# Autodesk Inventor assembly: FINGER_asm
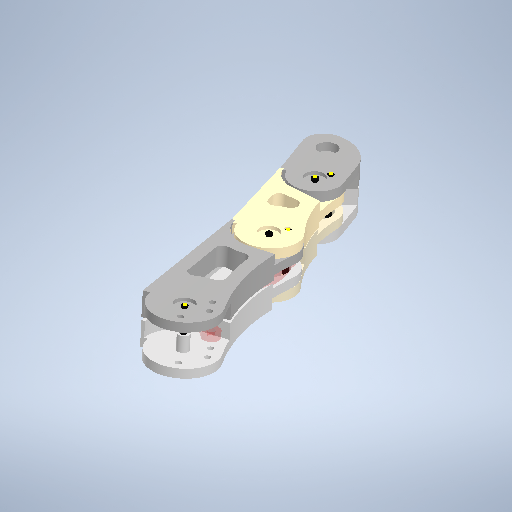
[picture p0: Inventor's stored thumbnail of the model, 512x512]
Saved by Autodesk Inventor 2025.2 (Build 292293000, 293)
## iProperties
Created: 2024-11-09
Part Number: FINGER_asm
Document SubType Name: Assembly
Designer: esandor
Author: esandor
## Documents named in this file (11)
- C:\Users\esandor\Documents\Inventor\Workspace\LEGO_GITHUB_INDACT_CAD\FINGER\FINGER_asm.iam
- C:\Users\esandor\Documents\Inventor\Workspace\LEGO_GITHUB_INDACT_CAD\FINGER\FIN_PD_B.ipt
- C:\Users\esandor\Documents\Inventor\Workspace\LEGO_GITHUB_INDACT_CAD\FINGER\FIN_PM_B.ipt
- C:\Users\esandor\Documents\Inventor\Workspace\LEGO_GITHUB_INDACT_CAD\FINGER\FIN_PP_B.ipt
- C:\Users\esandor\Documents\Inventor\Workspace\LEGO_GITHUB_INDACT_CAD\FINGER\FIN_PD_T.ipt
- C:\Users\esandor\Documents\Inventor\Workspace\LEGO_GITHUB_INDACT_CAD\FINGER\FIN_PM_T.ipt
- C:\Users\esandor\Documents\Inventor\Workspace\LEGO_GITHUB_INDACT_CAD\FINGER\FIN_DP_L.ipt
- C:\Users\esandor\Documents\Inventor\Workspace\LEGO_GITHUB_INDACT_CAD\FINGER\FIN_PP_T.ipt
- C:\Users\esandor\Documents\Inventor\Workspace\LEGO_GITHUB_INDACT_CAD\FINGER\FIN_DP_S.ipt
- C:\Users\esandor\Documents\Inventor\Workspace\LEGO_GITHUB_INDACT_CAD\FINGER\FIN_MD.ipt
- C:\Users\esandor\Documents\Inventor\Workspace\LEGO_GITHUB_INDACT_CAD\FINGER\FIN_MP.ipt
## Components (15 placed, 10 different names)
1. FIN_PD_B:1 — Mate:1, Rotational:1, Mate:3, Insert:1, Insert:2, Insert:5, Insert:9
2. FIN_PM_B:1 — Mate:1, Rotational:1, Insert:4, Rotational:2, Insert:10
3. FIN_PD_T:1 — Mate:3, Insert:1, Insert:2, Mate:4, Insert:3, Tangent:3
4. FIN_PM_T:1 — Mate:4, Insert:3, Tangent:1, Insert:6
5. FIN_DP_L:1 — Insert:4, Tangent:1
6. FIN_DP_L:2 — Insert:5, Insert:8
7. FIN_PP_B:1 — Rotational:2, Insert:7, Insert:11, Insert:12
8. FIN_PP_T:1 — Insert:6, Tangent:2, Mate:6, Tangent:6
9. FIN_DP_L:3 — Insert:7, Tangent:2
10. FIN_DP_L:4 — Insert:8
11. FIN_DP_L:6 — Insert:9, Tangent:3, Tangent:4
12. FIN_DP_L:7 — Insert:10, Tangent:5
13. FIN_DP_S:1 — Insert:11
14. FIN_MD:1 — Insert:12, Tangent:4
15. FIN_MP:1 — Tangent:5, Mate:6, Tangent:6
## Relationships (24: Insert 12, Tangent 6, Mate 4, RevoluteJoint 2)
- Mate:1: FIN_PD_B:1 ↔ FIN_PM_B:1
- Rotational:1 [RevoluteJoint]: FIN_PD_B:1 ↔ FIN_PM_B:1
- Mate:3: FIN_PD_B:1 ↔ FIN_PD_T:1
- Insert:1: FIN_PD_B:1 ↔ FIN_PD_T:1
- Insert:2: FIN_PD_B:1 ↔ FIN_PD_T:1
- Mate:4: FIN_PD_T:1 ↔ FIN_PM_T:1
- Insert:3: FIN_PD_T:1 ↔ FIN_PM_T:1
- Insert:4 (-0.8 mm): FIN_PM_B:1 ↔ FIN_DP_L:1
- Tangent:1: FIN_PM_T:1 ↔ FIN_DP_L:1
- Insert:5 (-1 mm): FIN_PD_B:1 ↔ FIN_DP_L:2
- Rotational:2 [RevoluteJoint]: FIN_PM_B:1 ↔ FIN_PP_B:1
- Insert:6: FIN_PM_T:1 ↔ FIN_PP_T:1
- Insert:7 (-0.6 mm): FIN_PP_B:1 ↔ FIN_DP_L:3
- Tangent:2: FIN_PP_T:1 ↔ FIN_DP_L:3
- Insert:8: FIN_DP_L:2 ↔ FIN_DP_L:4
- Insert:9: FIN_PD_B:1 ↔ FIN_DP_L:6
- Tangent:3: FIN_PD_T:1 ↔ FIN_DP_L:6
- Insert:10 (0.2 mm): FIN_PM_B:1 ↔ FIN_DP_L:7
- Insert:11: FIN_PP_B:1 ↔ FIN_DP_S:1
- Insert:12: FIN_PP_B:1 ↔ FIN_MD:1
- Tangent:4: FIN_DP_L:6 ↔ FIN_MD:1
- Tangent:5: FIN_DP_L:7 ↔ FIN_MP:1
- Mate:6: FIN_PP_T:1 ↔ FIN_MP:1
- Tangent:6: FIN_PP_T:1 ↔ FIN_MP:1
